# Autodesk Inventor assembly: Stewart-Base-KST-DS215
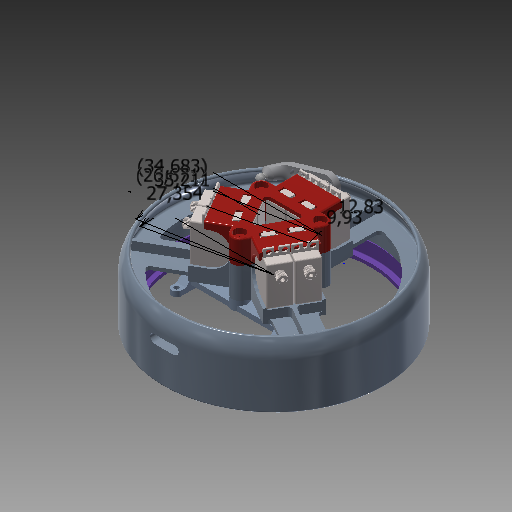
[picture p0: Inventor's stored thumbnail of the model, 512x512]
Saved by Autodesk Inventor 2018.3 (Build 223284000, 284)
## iProperties
Created: 2018-02-24
Part Number: Stewart-Base-KST-DS215
Material: Generisch
Document SubType Name: Assembly
Designer: JochenAlt
Author: JochenAlt
## Documents named in this file (5)
- D:\Projects\Donna\CAD\Stewart-Base.iam
- D:\Projects\Donna\CAD\Servo-KST-DS215MG.ipt
- D:\Projects\Donna\CAD\Messung.ipt
- D:\Projects\Donna\CAD\Servo-Arm-Head-20mm-Ball-Joint.iam
- D:\Projects\Donna\CAD\Stewart-Platform-Base.ipt
## Components (9 placed, 4 different names)
1. Servo-KST-DS215MG:1 — Passend:70, Passend:84, Passend:86
2. Servo-KST-DS215MG:2 — Passend:69, Passend:83, Passend:85
3. Servo-KST-DS215MG:3 — Passend:72, Passend:80, Passend:82
4. Servo-KST-DS215MG:4 — Passend:71, Passend:79, Passend:81
5. Servo-KST-DS215MG:5 — Passend:74, Passend:76, Passend:77
6. Servo-KST-DS215MG:6 — Passend:67, Passend:68, Passend:73, Passend:75, Passend:78
7. Servo-Arm-Head-20mm-Ball-Joint:1 [sub-assembly] — Passend:67, Passend:68
8. Messung:1 — Fluchtend:1
9. Stewart-Platform-Base:1 — Passend:69, Passend:70, Passend:71, Passend:72, Passend:73, Passend:74, Passend:75, Passend:76, Passend:77, Passend:78, Passend:79, Passend:80, Passend:81, Passend:82, Passend:83, Passend:84, Passend:85, Passend:86
## Relationships (21: Mate 20, Flush 1)
- Fluchtend:1 [Flush]: Messung:1
- Passend:67 [Mate]: Servo-KST-DS215MG:6 ↔ Servo-Arm-Head-20mm-Ball-Joint:1
- Passend:68 [Mate]: Servo-KST-DS215MG:6 ↔ Servo-Arm-Head-20mm-Ball-Joint:1
- Passend:69 [Mate]: Servo-KST-DS215MG:2 ↔ Stewart-Platform-Base:1
- Passend:70 [Mate]: Servo-KST-DS215MG:1 ↔ Stewart-Platform-Base:1
- Passend:71 [Mate]: Servo-KST-DS215MG:4 ↔ Stewart-Platform-Base:1
- Passend:72 [Mate]: Servo-KST-DS215MG:3 ↔ Stewart-Platform-Base:1
- Passend:73 [Mate]: Servo-KST-DS215MG:6 ↔ Stewart-Platform-Base:1
- Passend:74 [Mate]: Servo-KST-DS215MG:5 ↔ Stewart-Platform-Base:1
- Passend:75 [Mate]: Servo-KST-DS215MG:6 ↔ Stewart-Platform-Base:1
- Passend:76 [Mate]: Servo-KST-DS215MG:5 ↔ Stewart-Platform-Base:1
- Passend:77 [Mate]: Servo-KST-DS215MG:5 ↔ Stewart-Platform-Base:1
- Passend:78 [Mate]: Servo-KST-DS215MG:6 ↔ Stewart-Platform-Base:1
- Passend:79 [Mate]: Servo-KST-DS215MG:4 ↔ Stewart-Platform-Base:1
- Passend:80 [Mate]: Servo-KST-DS215MG:3 ↔ Stewart-Platform-Base:1
- Passend:81 [Mate]: Servo-KST-DS215MG:4 ↔ Stewart-Platform-Base:1
- Passend:82 [Mate]: Servo-KST-DS215MG:3 ↔ Stewart-Platform-Base:1
- Passend:83 [Mate]: Servo-KST-DS215MG:2 ↔ Stewart-Platform-Base:1
- Passend:84 [Mate]: Servo-KST-DS215MG:1 ↔ Stewart-Platform-Base:1
- Passend:85 [Mate]: Servo-KST-DS215MG:2 ↔ Stewart-Platform-Base:1
- Passend:86 [Mate]: Servo-KST-DS215MG:1 ↔ Stewart-Platform-Base:1
